# Autodesk Inventor assembly: 015.5-P(F,D-850)
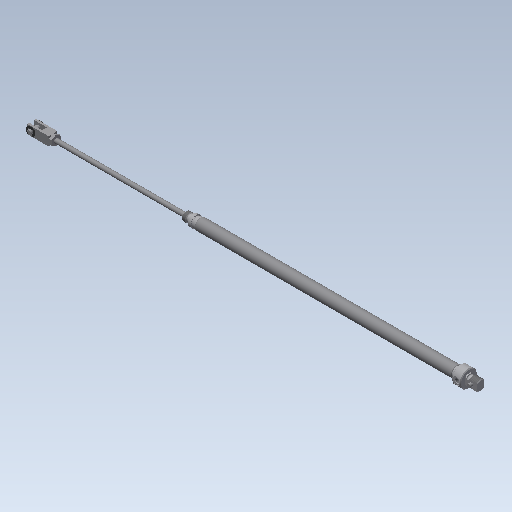
[picture p0: Inventor's stored thumbnail of the model, 512x512]
Saved by Autodesk Inventor 2020 (Build 240168000, 168)
## iProperties
Created: 2020-01-07
Part Number: 015.5-P(F,D-850)
Catalog Web Link: www.cadenas.de
Description: Original Line Standard Air Cylinders-Standard Air Cylinders
Vendor: BIMBA
Document SubType Name: Assembly
Designer: psadmin
Manufacturer: BIMBA
Category: PARTsolutions
Company: BIMBA
PSOL_IDENT_0: {$CADENAS_DATA\23d-libs\bimba\bimba_brand\bimba_imperial\bimba_full_line\original_line_cylinders\sta
PSOL_IDENT_1: ndard_air_cylinders\standard_air_cylinder_asmtab.prj},331 {VTYP=3D},{STYP=ASSTAB},{NB=015.5-P(F,D-85
PSOL_IDENT_2: 0)},{LINA=015.5-P},{NN=Original Line Standard Air Cylinders},{DATE=23.12.2019 10:36:48},{GEOMDATE=24
PSOL_IDENT_3: .10.2019 09:09:47},{VERSION=},{LINEID=30},{WBVAR=STROKE,ACTING,MNT,DER,NR,BM,CO,OO,VO,M,EE,EEL,K,Q,Y
PSOL_IDENT_4: ,G,T,HL,B,H,SER,SR,NT,W,STPT1,STPT2,STPT3,STPT4,MB,PB,PRC,TB,MN},{WBNUMERIC=STROKE,EEL}  {NB=015.5-P
PSOL_IDENT_5: (F,D-850)},{LINA=015.5-P},{KT=DUMMY},{PN=015.5-P},{PNC=015.5-P(F,D-850)},{PNA=(D-850)},{DASH=-},{BOR
PSOL_IDENT_6: E1=0.43750000},{BORE=7/16\" (01)},{BOREPN=01},{STROKE=5.500},{STROKEALG=[0.011:50/0.001]},{STROKE1=5
PSOL_IDENT_7: .500},{ACTING=},{ACTINGALG= '' , 'Single Acting' , 'R' , 'Reverse Single Acting (R)' , 'D' , 'Double
PSOL_IDENT_8: Acting (D)' },{ACTINGPN=},{MNT=P},{MNTALG= '' , 'Front Nose Mounting' , 'P' , 'Rear Pivot Mounting
PSOL_IDENT_9: (P)' , 'BF' , 'Front Block Mounting (BF)' , 'BR' , 'Rear Block Mounting for Vertical Positioning (BR
PSOL_IDENT_10: )' , 'BFT' , 'Front Block Trunnion Mounting (BFT)' , 'BRT' , 'Rear Block Trunnion Mounting (BRT)' },
PSOL_IDENT_11: {TYPE=},{MNTPN=P},{DER=},{DERALG= '' , 'N/A' },{NR=},{NRALG= '' , 'Round (Standard)' , 'NR' , 'Non-r
PSOL_IDENT_12: otating - Hexagon Rod' },{NRPN=},{BM=},{BMALG= '' , 'N/A' },{BMPN=},{CO=},{COALG= '' , 'N/A' },{OO=}
PSOL_IDENT_13: ,{OOALG= '', 'N/A' },{OOPN=},{VO=Z},{VOALG= 'Z' , 'N/A' },{VOPN=},{OOVOPN=},{M=},{MALG= '', 'Without
PSOL_IDENT_14: Magnet', 'M', 'With Magnet' },{EE=},{EEL=0.000},{EEMAX=44.5000},{EEALG= '', 'Without Extra Extensio
PSOL_IDENT_15: n', 'EE', 'With Extra Extension' },{EELALG=0},{EEPN=},{EEPN1=0.000},{K=},{KALG= '', 'Standard' , 'K'
PSOL_IDENT_16: , 'Ports Rotated 90deg K' },{KPN=},{Q=},{QALG= '' , 'N/A' },{QPN=},{Y=},{YALG= '' , 'Without Pivot
PSOL_IDENT_17: Bushing' , 'Y' , 'With Pivot Bushing' },{YPN=},{YCON=},{F=},{FALG= '', 'Non-Coated (Standard)', 'F',
PSOL_IDENT_18: 'Molycoated' },{FPN=},{G=},{GPN=},{GPN99=},{T=},{TALG= '' , 'Standard -20° to 200°F (-29° to 95°C)'
PSOL_IDENT_19: , 'N' , 'Low Temperature' , 'V' , 'High Temperature' },{NPN=},{VPN=},{HL=},{HLALG= '' , 'N/A' },{B=
PSOL_IDENT_20: },{BALG= '', 'W/out Bumpers' , 'B' , 'W/ Bumpers' },{BPN=},{H=},{HALG= '', 'N/A' },{HPN=},{SER=},{SE
PSOL_IDENT_21: RALG= '' , 'N/A' },{SR=},{SRALG= '' , 'Standard Stainless Steel' },{SRPN=},{SRCON=0},{NT=},{NTPN=},{
PSOL_IDENT_22: W=},{WALG= '' , 'N/A' },{WPN=},{E=},{EALG= '' , 'Standard Seals/Lube' , 'E' , 'Non-Lube Seals/Lube'
PSOL_IDENT_23: },{EPN=},{ST=},{STALG= '' , 'N/A' },{STPT1=},{STPT1ALG= '' , 'N/A' },{STPT2=},{STPT2ALG= '' , 'N/A'
PSOL_IDENT_24: },{STPT3=},{STPT3ALG= '' , 'N/A' },{STPT4=},{STPT4ALG= '' , 'N/A' },{STPN=},{MB=},{MBALG= '' , 'N/A'
PSOL_IDENT_25: },{MBPN=},{MBPNALL=},{MBPNALLREAR=},{PB=},{PBALG= '' , 'Without Pivot Bracket' , 'D-780' , 'D-780'
PSOL_IDENT_26: },{PBPN=},{PBPNALL=D-780},{PRC=F,D-850},{PRCALG= '' , 'W/out Pivot Rod Clevis' , 'F,D-850' , 'D-850
PSOL_IDENT_27: (front)' },{PRCPN=(F,D-850)},{PRCPNALL=D-850},{TB=},{TBALG= '' , 'N/A' },{TBPN=},{TBPNALL=},{MN=},{M
PSOL_IDENT_28: NALG= '' , 'Without Mounting Nut' , 'F,D-801' , 'D-801 (front)' , 'R,D-154' , 'D-154 (rear)', '2xZ'
PSOL_IDENT_29: , 'D-801 (front) & D-154 (rear)' },{MNPN=},{MNCONF=},{MNCONR=},{TLEN=10.8620},{FRAC=12.0900},{RGCON=
PSOL_IDENT_30: },{RGDACCON=},{RHCON=P},{RHCON1=P},{RHCONON=1},{RHACCON=},{FNUTCON=0},{RNUTCON=0},{FNUTPN=D-801},{RN
PSOL_IDENT_31: UTPN=D-154},{FNUTTRANS=0.0000},{RNUTTRANS=0.0000},{VHOLECON=2},{A1=0.6880},{A1N=0.6880},{A1P=1.1880}
PSOL_IDENT_32: ,{A1B=1.1880},{A4=0.2500},{A4N=0.2500},{A4P=0.1880},{A5=0.0200},{A1H=1.188},{A1NH=0.5000},{A1PH=1.18
PSOL_IDENT_33: 80},{A1BH=0.8120},{A1SH=0.0000},{A2H=0.1880},{A2NH=0.1880},{LENGTH=1.7500},{LENGTH1=1.7500},{LENGTH2=
PSOL_IDENT_34: 2.6100},{MUL=10.3400},{MUL11=10.3400},{MUL22=15.84},{MUL33=10.3400},{MUL2=0.9400},{MUL211=0.9400},{M
PSOL_IDENT_35: UL222=1.4400},{MUL233=0.9400},{SSS=11.0000},{RGLEN=0.4580},{RHLEN=0.7700},{SSS1=11.0000},{A13=0.9380
PSOL_IDENT_36: },{DIF=0.0000},{G5=0.0000},{ON=0},{SSADD=0.0000},{BADD=0.0000},{MADD=0.0000},{NVADD=0.0000},{TRACKL=
PSOL_IDENT_37: 10.5520},{TRACKCON=D-74168},{TRIMCON=0},{TRIMCON1=0},{PINCON=D-787},{FSPACE=0.3608},{SPACE=0.0594},{
PSOL_IDENT_38: TEXT=0.1039},{S1=0.7500},{D1=0.4840},{D1N=0.4840},{D1B=0.7380},{D1P=0.0000},{FA=0.560},{RA=0.5600},{
PSOL_IDENT_39: PPATH=standard_air_cylinder_asmtpl.prj},{MATALGHTML=<b>Standard Original Line:</b><dl><dt>Rod:</dt><
PSOL_IDENT_40: dd>- Stainless Steel</dd><dd>&nbsp;&nbsp;(5/16 9/16 Bores)</dd><dd>- High Strength Carbon Steel</dd>
PSOL_IDENT_41: <dd>&nbsp;&nbsp;(3/4 3 Bore)</dd><dd>- Stainless Steel</dd><dd>&nbsp;&nbsp;(X style DXP/DX/DXDE)</dd
PSOL_IDENT_42: ><dt>Bearings:</dt><dd>- Sintered Bronze</dd><dt>Body:</dt><dd>- 304 Stainless Steel</dd><dt>End Cap
PSOL_IDENT_43: s:</dt><dd>- Aluminum</dd><dt>Seals:</dt><dd>- Buna N</dd></dl>},{ASSCFGPRA=01P},{MBPNA=},{MNPNA=},{
PSOL_IDENT_44: PRCPNA=(D-850)},{ASSOPTACC=STPT4},{A=12.09},{HADD=0.0000},{WFL=0},{QADD=0.000},{QADD1=0.190},{TEST=5
PSOL_IDENT_45: .0000},{MNTB=},{STDNUTF=0},{STDNUTR=0},{STRK2D=0},{X2D=2},{STROKESW=5.500},{EESW=0.000},{FCD=0},{BCD=
PSOL_IDENT_46: 0},{RCD=0},{CUSTADD=4.500},{FT=#10-32 UNF-2A},{FT1=#10-32 UNF-2A},{FT2=7/16-20 UNF-2A},{PORT=#10-32}
PSOL_IDENT_47: ,{FT11=3/8-24 UNF-2A},{FT12=7/16-20 UNF-2A},{B1=}
NN: Original Line Standard Air Cylinders
NT: Threaded (Standard)
NB: 015.5-P(F,D-850)
NBSYN: $PNC.
LINA: 015.5-P
PN: 015.5-P
PNA: (D-850)
BORE: 7/16" (01)
STROKE: 5.5
ACTING: Single [Standard]
MNT: Rear Pivot Mounting (P)
DER: N/A
NR: Round (Standard)
BM: N/A
CO: N/A
OO: N/A
VO: N/A
M: Without Magnet
EE: Without Extra Extension
EEL: 0
K: Standard
Q: N/A
Y: Without Pivot Bushing
G: Standard Lube
T: Standard -20° to 200°F (-29° to 95°C)
HL: N/A
B: W/out Bumpers
H: N/A
SER: N/A
SR: Standard Stainless Steel
W: N/A
STPT1: N/A
STPT2: N/A
STPT3: N/A
STPT4: N/A
MB: N/A
PB: Without Pivot Bracket
PRC: D-850 (front)
TB: N/A
MN: Without Mounting Nut
A: 12.09
SUPPLIER: BIMBA
ARTICLENO: 015.5-P(F,D-850)
BOMINFO: 015.5-P
CREATOR: CADENAS GmbH
Title: 015.5-P
Author: Cadenas PARTsolutions
Comments: Standard Air Cylinders
## Documents named in this file (12)
- D:\My Docs\Robotics\Robot Stuff\STEP Files\Pnumatics\5.5inExt_7-16in Boar\PARTserver0202001070223121533149410e898ce\AIS2018\015_5-P(F,D-850).iam
- D:\My Docs\Robotics\Robot Stuff\STEP Files\Pnumatics\5.5inExt_7-16in Boar\PARTserver0202001070223121533149410e898ce\AIS2018\015_5-P(F,D-850)0000000_0_dummy.ipt
- D:\My Docs\Robotics\Robot Stuff\STEP Files\Pnumatics\5.5inExt_7-16in Boar\PARTserver0202001070223121533149410e898ce\AIS2018\01000-0_rod_guide.ipt
- D:\My Docs\Robotics\Robot Stuff\STEP Files\Pnumatics\5.5inExt_7-16in Boar\PARTserver0202001070223121533149410e898ce\AIS2018\01-10_8622.ipt
- D:\My Docs\Robotics\Robot Stuff\STEP Files\Pnumatics\5.5inExt_7-16in Boar\PARTserver0202001070223121533149410e898ce\AIS2018\01P0000_rear_head.ipt
- D:\My Docs\Robotics\Robot Stuff\STEP Files\Pnumatics\5.5inExt_7-16in Boar\PARTserver0202001070223121533149410e898ce\AIS2018\D-787.ipt
- D:\My Docs\Robotics\Robot Stuff\STEP Files\Pnumatics\5.5inExt_7-16in Boar\PARTserver0202001070223121533149410e898ce\AIS2018\015_5-P0000_rod.ipt
- D:\My Docs\Robotics\Robot Stuff\STEP Files\Pnumatics\5.5inExt_7-16in Boar\PARTserver0202001070223121533149410e898ce\AIS2018\D-850-dummy.ipt
- D:\My Docs\Robotics\Robot Stuff\STEP Files\Pnumatics\5.5inExt_7-16in Boar\PARTserver0202001070223121533149410e898ce\AIS2018\D-14043.ipt
- D:\My Docs\Robotics\Robot Stuff\STEP Files\Pnumatics\5.5inExt_7-16in Boar\PARTserver0202001070223121533149410e898ce\AIS2018\D-12304.ipt
- D:\My Docs\Robotics\Robot Stuff\STEP Files\Pnumatics\5.5inExt_7-16in Boar\PARTserver0202001070223121533149410e898ce\AIS2018\D-5406.ipt
- D:\My Docs\Robotics\Robot Stuff\STEP Files\Pnumatics\5.5inExt_7-16in Boar\PARTserver0202001070223121533149410e898ce\AIS2018\D-5288.ipt
## Components (12 placed, 11 different names)
1. 015_5-P(F,D-850)0000000_0_dummy:1
2. 01000-0_rod_guide:1 — Mate:4, Mate:5, Mate:6, Mate:7
3. 01-10_8622:1 — Mate:2, Mate:3, Mate:4, Mate:5
4. 01P0000_rear_head:1 — Mate:1, Flush:1, Mate:2, Mate:3
5. D-787:1 — Mate:1, Flush:1
6. 015_5-P0000_rod:1 — Mate:6
7. D-850-dummy:1
8. D-14043:1
9. D-12304:1
10. D-5406:1
11. D-5406:2
12. D-5288:1 — Mate:7
## Relationships (8: Mate 7, Flush 1)
- Mate:1: 01P0000_rear_head:1 ↔ D-787:1
- Flush:1 (-2.54 mm): 01P0000_rear_head:1 ↔ D-787:1
- Mate:2: 01-10_8622:1 ↔ 01P0000_rear_head:1
- Mate:3: 01-10_8622:1 ↔ 01P0000_rear_head:1
- Mate:4: 01000-0_rod_guide:1 ↔ 01-10_8622:1
- Mate:5: 01000-0_rod_guide:1 ↔ 01-10_8622:1
- Mate:6: 01000-0_rod_guide:1 ↔ 015_5-P0000_rod:1
- Mate:7 (139.7 mm): 01000-0_rod_guide:1 ↔ D-5288:1
